# Autodesk Inventor assembly: motor assembly
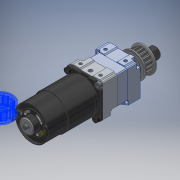
[picture p0: Inventor's stored thumbnail of the model, 180x180]
Saved by Autodesk Inventor 2018 (Build 220112000, 112)
## iProperties
Created: 2019-02-24
Part Number: motor assembly
Document SubType Name: Assembly
Designer: Tiberus
Author: Tiberus
## Documents named in this file (3)
- \\studenthome\students\S-2513225\GitHub\2019CAD\NEW NEW GRIPPER (feb 23)\motor assembly.iam
- \\studenthome\students\S-2513225\GitHub\2019CAD\NEW NEW GRIPPER (feb 23)\VersaPlanetary_v2_Single_Stage_10_1_with_775_Series.ipt
- \\studenthome\students\S-2513225\GitHub\2019CAD\NEW NEW GRIPPER (feb 23)\18t_x_9mm_Wide_Double_Flange_Aluminum_Pulley_HTD_5mm_1_2_Hex_Bore_217-3225.ipt
## Components (2 placed, 2 different names)
1. VersaPlanetary_v2_Single_Stage_10_1_with_775_Series:1 — Mate:1, Mate:2, Mate:3
2. 18t_x_9mm_Wide_Double_Flange_Aluminum_Pulley_HTD_5mm_1_2_Hex_Bore_217-3225:1 — Mate:1, Mate:2, Mate:3
## Relationships (3: Mate 3)
- Mate:1: VersaPlanetary_v2_Single_Stage_10_1_with_775_Series:1 ↔ 18t_x_9mm_Wide_Double_Flange_Aluminum_Pulley_HTD_5mm_1_2_Hex_Bore_217-3225:1
- Mate:2: VersaPlanetary_v2_Single_Stage_10_1_with_775_Series:1 ↔ 18t_x_9mm_Wide_Double_Flange_Aluminum_Pulley_HTD_5mm_1_2_Hex_Bore_217-3225:1
- Mate:3: VersaPlanetary_v2_Single_Stage_10_1_with_775_Series:1 ↔ 18t_x_9mm_Wide_Double_Flange_Aluminum_Pulley_HTD_5mm_1_2_Hex_Bore_217-3225:1
